# Autodesk Inventor assembly: Metal Scoop Breakable
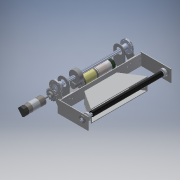
[picture p0: Inventor's stored thumbnail of the model, 180x180]
Saved by Autodesk Inventor 2017 (Build 210142000, 142)
## iProperties
Created: 2017-06-10
Part Number: Metal Scoop Breakable
Document SubType Name: Assembly
Designer: Matthew
Author: Matthew
## Documents named in this file (20)
- C:\Inventor Stuff\Robotics Trash\Metal Scoop\Metal Scoop Breakable.iam
- C:\Inventor Stuff\Robotics Trash\Metal Scoop\Top + Bottom.ipt
- C:\Inventor Stuff\Robotics Trash\Metal Scoop\Back Wall.ipt
- C:\Inventor Stuff\Robotics Trash\Metal Scoop\Side Wall.ipt
- C:\Inventor Stuff\Robotics Trash\Metal Scoop\Top + Spinner.ipt
- C:\Inventor Stuff\Robotics Trash\VexPro 15 Tooth Sprocket.ipt
- C:\Inventor Stuff\Robotics Trash\Metal Scoop\Pivot Bracket 2.ipt
- C:\Inventor Stuff\Robotics Trash\FRC Yellow Gear.iam
- C:\Inventor Stuff\Robotics Trash\Metal Scoop\3in PD Gear.ipt
- C:\Inventor Stuff\Robotics Trash\Metal Scoop\1in PD Gear.ipt
- C:\Inventor Stuff\Robotics Trash\PG 188 + Encoder.iam
- C:\Inventor Stuff\Robotics Trash\Churro Clamp.iam
- C:\Inventor Stuff\Robotics Trash\Churro.ipt
- C:\Inventor Stuff\Robotics Trash\Bearing.ipt
- C:\Inventor Stuff\Robotics Trash\Metal Scoop\New Roller.ipt
- C:\Inventor Stuff\Robotics Trash\Metal Scoop\16 Tooth Sprocket.ipt
- C:\Inventor Stuff\Robotics Trash\Tetrix Neverest 20 Motor.ipt
- C:\Inventor Stuff\Robotics Trash\Hex Hub.ipt
- C:\Inventor Stuff\Robotics Trash\PG Motor Bracket.ipt
- C:\Inventor Stuff\Robotics Trash\Metal Scoop\Another Motor Bracket.ipt
## Components (26 placed, 19 different names)
1. Top + Bottom:1 — Mate:2, Flush:2, Mate:11, Mate:17, Flush:10, Mate:18, Mate:19, Flush:11, Mate:53
2. Back Wall:1 — Mate:2, Flush:2, Mate:11, Flush:12, Mate:21, Mate:28
3. Side Wall:1 — Mate:17, Flush:10, Mate:18, Mate:22
4. Side Wall:2 — Mate:19, Flush:11
5. Top + Spinner:1 — Flush:12, Mate:21, Mate:22, Flush:15
6. VexPro 15 Tooth Sprocket:2 — Mate:75, Flush:18, Mate:91
7. Pivot Bracket 2:1 — Mate:28, Flush:15, Mate:65, Mate:66, Mate:68, Mate:69, Mate:80, Mate:81, Mate:85, Mate:86, Mate:87, Mate:88, Mate:91, Mate:92, Mate:93, Mate:95
8. FRC Yellow Gear:1 [sub-assembly] — Mate:53
9. 3in PD Gear:1 — Flush:16, Tangent:1, Mate:92
10. 1in PD Gear:1 — Flush:16, Mate:57, Flush:17, Tangent:1, Mate:94
11. PG 188 + Encoder:1 [sub-assembly] — Mate:57, Flush:17, Mate:98, Mate:99
12. Churro Clamp:1 [sub-assembly] — Mate:71
13. Churro:1 — Mate:62, Mate:63, Mate:70, Flush:20
14. Churro:2 — Mate:62, Mate:63, Flush:19
15. Bearing:1 — Mate:65, Mate:68, Mate:70, Mate:71, Mate:73, Flush:20
16. Bearing:2 — Mate:66, Mate:69, Flush:19
17. New Roller:1 — Mate:73, Mate:74, Mate:77
18. 16 Tooth Sprocket:1 — Mate:74, Flush:18
19. Tetrix Neverest 20 Motor:1 — Mate:75
20. Churro Clamp:3 [sub-assembly] — Mate:77
21. Churro:3 — Mate:90, Flush:21, Flush:22, Mate:93
22. Hex Hub:1 — Mate:81, Mate:85, Mate:87, Mate:90
23. Hex Hub:2 — Mate:80, Mate:86, Mate:88, Mate:96
24. Churro:4 — Flush:21, Flush:22
25. PG Motor Bracket:1 — Mate:94, Mate:97, Mate:98, Mate:99, Mate:100, Mate:101
26. Another Motor Bracket:1 — Mate:95, Mate:96, Mate:97, Mate:100, Mate:101
## Relationships (53: Mate 40, Flush 12, Tangent 1)
- Mate:2: Top + Bottom:1 ↔ Back Wall:1
- Flush:2: Top + Bottom:1 ↔ Back Wall:1
- Mate:11: Top + Bottom:1 ↔ Back Wall:1
- Mate:17: Top + Bottom:1 ↔ Side Wall:1
- Flush:10: Top + Bottom:1 ↔ Side Wall:1
- Mate:18: Top + Bottom:1 ↔ Side Wall:1
- Mate:19: Top + Bottom:1 ↔ Side Wall:2
- Flush:11: Top + Bottom:1 ↔ Side Wall:2
- Flush:12: Back Wall:1 ↔ Top + Spinner:1
- Mate:21: Back Wall:1 ↔ Top + Spinner:1
- Mate:22: Side Wall:1 ↔ Top + Spinner:1
- Mate:28: Back Wall:1 ↔ Pivot Bracket 2:1
- Flush:15 (-12.7 mm): Top + Spinner:1 ↔ Pivot Bracket 2:1
- Mate:53: Top + Bottom:1 ↔ FRC Yellow Gear:1
- Flush:16 (-3.175 mm): 3in PD Gear:1 ↔ 1in PD Gear:1
- Mate:57: 1in PD Gear:1 ↔ PG 188 + Encoder:1
- Flush:17 (6.35 mm): 1in PD Gear:1 ↔ PG 188 + Encoder:1
- Mate:62: Churro:1 ↔ Churro:2
- Mate:63: Churro:1 ↔ Churro:2
- Mate:65: Pivot Bracket 2:1 ↔ Bearing:1
- Mate:66: Pivot Bracket 2:1 ↔ Bearing:2
- Mate:68: Pivot Bracket 2:1 ↔ Bearing:1
- Mate:69: Pivot Bracket 2:1 ↔ Bearing:2
- Mate:70: Churro:1 ↔ Bearing:1
- Mate:71: Churro Clamp:1 ↔ Bearing:1
- Mate:73: Bearing:1 ↔ New Roller:1
- Mate:74: New Roller:1 ↔ 16 Tooth Sprocket:1
- Mate:75: VexPro 15 Tooth Sprocket:2 ↔ Tetrix Neverest 20 Motor:1
- Flush:18: VexPro 15 Tooth Sprocket:2 ↔ 16 Tooth Sprocket:1
- Mate:77: New Roller:1 ↔ Churro Clamp:3
- Mate:80: Pivot Bracket 2:1 ↔ Hex Hub:2
- Mate:81: Pivot Bracket 2:1 ↔ Hex Hub:1
- Flush:19 (-6.35 mm): Churro:2 ↔ Bearing:2
- Flush:20 (-6.35 mm): Churro:1 ↔ Bearing:1
- Mate:85: Pivot Bracket 2:1 ↔ Hex Hub:1
- Mate:86: Pivot Bracket 2:1 ↔ Hex Hub:2
- Mate:87: Pivot Bracket 2:1 ↔ Hex Hub:1
- Mate:88: Pivot Bracket 2:1 ↔ Hex Hub:2
- Mate:90 (0.0254 mm): Churro:3 ↔ Hex Hub:1
- Mate:91: VexPro 15 Tooth Sprocket:2 ↔ Pivot Bracket 2:1
- Tangent:1: 3in PD Gear:1 ↔ 1in PD Gear:1
- Flush:21: Churro:3 ↔ Churro:4
- Flush:22: Churro:3 ↔ Churro:4
- Mate:92: Pivot Bracket 2:1 ↔ 3in PD Gear:1
- Mate:93: Pivot Bracket 2:1 ↔ Churro:3
- Mate:94: 1in PD Gear:1 ↔ PG Motor Bracket:1
- Mate:95: Pivot Bracket 2:1 ↔ Another Motor Bracket:1
- Mate:96 (10.414 mm): Hex Hub:2 ↔ Another Motor Bracket:1
- Mate:97: PG Motor Bracket:1 ↔ Another Motor Bracket:1
- Mate:98: PG 188 + Encoder:1 ↔ PG Motor Bracket:1
- Mate:99: PG 188 + Encoder:1 ↔ PG Motor Bracket:1
- Mate:100: PG Motor Bracket:1 ↔ Another Motor Bracket:1
- Mate:101: PG Motor Bracket:1 ↔ Another Motor Bracket:1
